# Autodesk Inventor assembly: Assembly2
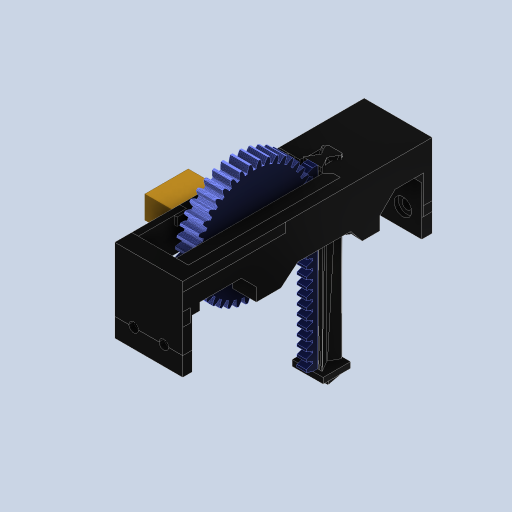
[picture p0: Inventor's stored thumbnail of the model, 512x512]
Saved by Autodesk Inventor 2023.1 (Build 271208000, 208)
## iProperties
Created: 2024-08-02
Part Number: Assembly2
Document SubType Name: Assembly
Designer: huchonms
Engineer: vikt
Mass: 921.395 g
Surface Area: 435.625 cm^2
Volume: 117.375 cm^3
Density: 7.85 g/cm^3
tc_part_rev_length: 70
tc_part_rev_width: 132
tc_part_rev_height: 152
tc_part_rev_uom_length: mm
tc_part_rev_volume: 117375
tc_part_rev_uom_volume: mm^3
tc_part_rev_mass: 0.92
tc_part_rev_uom_mass: kg
NOV_FileName: Assembly2
Author: huchonms
Revision Number: 0
## Documents named in this file (5)
- C:\VaultWork\Designs\_Scratch_\Marius Huchon\Sommerprosjekt_filer\Heis deler\Actuator_Servo\Inventor\Assembly2.iam
- C:\VaultWork\Designs\_Scratch_\Marius Huchon\Sommerprosjekt_filer\Heis deler\Actuator_Servo\Inventor\Spur_gear.ipt
- C:\VaultWork\Designs\_Scratch_\Marius Huchon\Sommerprosjekt_filer\Heis deler\Actuator_Servo\Inventor\Housing.ipt
- C:\VaultWork\Designs\_Scratch_\Marius Huchon\Sommerprosjekt_filer\Heis deler\Actuator_Servo\Inventor\Rack_assembly.iam
- C:\VaultWork\Designs\_Scratch_\Marius Huchon\Sommerprosjekt_filer\Heis deler\Actuator_Servo\Inventor\Servo.ipt
## Components (4 placed, 4 different names)
1. Housing:1 — Mate:1, Rotational:1, Mate:2, Mate:3
2. Rack_assembly:1 [sub-assembly] — Mate:1
3. Spur_gear:1 — Rotational:1
4. Servo:1 — Mate:2, Mate:3
## Relationships (4: Mate 3, RevoluteJoint 1)
- Mate:1: Housing:1 ↔ Rack_assembly:1
- Rotational:1 [RevoluteJoint]: Housing:1 ↔ Spur_gear:1
- Mate:2: Housing:1 ↔ Servo:1
- Mate:3: Housing:1 ↔ Servo:1
